# Autodesk Inventor assembly: Z Axis Bed Carrier Assembly
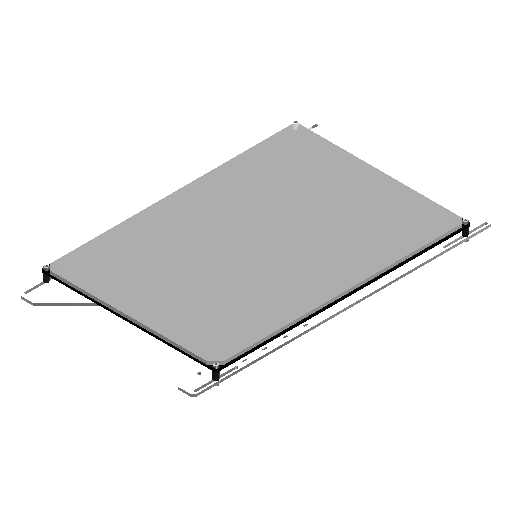
[picture p0: Inventor's stored thumbnail of the model, 512x512]
Saved by Autodesk Inventor 2023.2 (Build 272271000, 271)
## iProperties
Created: 2023-02-18
Part Number: Z Axis Bed Carrier Assembly
Document SubType Name: Assembly
Designer: remop
Author: remop
## Documents named in this file (7)
- C:\Users\remop\OneDrive\Documents\Inventor\3D Printers\LuEVO\Mk5_FullKinematic\Z Axis v2\Z Axis Bed Carrier Assembly.iam
- C:\Users\remop\OneDrive\Documents\Inventor\3D Printers\LuEVO\Mk5_FullKinematic\Z Axis v2\E3D High Temperature Bed 300x200.ipt
- C:\Users\remop\OneDrive\Documents\Inventor\3D Printers\LuEVO\Mk5_FullKinematic\Z Axis v2\Heated Bed Glass.ipt
- C:\Users\remop\OneDrive\Documents\Inventor\3D Printers\LuEVO\Mk5_FullKinematic\Z Axis v2\Bed Carrier.ipt
- C:\Users\remop\OneDrive\Documents\Inventor\3D Printers\LuEVO\Mk5_FullKinematic\Z Axis v2\Heated Bed Spacer.ipt
- C:\Users\remop\OneDrive\Documents\Inventor\3D Printers\LuEVO\Mk5_FullKinematic\XY Motion System\Toolhead\MagToolChanger_CouplerBall.ipt
- C:\Users\remop\OneDrive\Documents\Inventor\Content Center Files\R2023\en-US\AS 1420\AS 1420 - 1973 - M3 x 8.ipt
## Components (18 placed, 6 different names)
1. E3D High Temperature Bed 300x200:1 — Rigid:1, Mate:1, Rigid:2, Rigid:3, Rigid:4, Rigid:5, Insert:1, Insert:2, Insert:6, Insert:8
2. Heated Bed Glass:1 — Rigid:1
3. Bed Carrier:1 — Mate:1, Rigid:6, Rigid:7, Rigid:8
4. Heated Bed Spacer:1 — Rigid:4
5. Heated Bed Spacer:2 — Rigid:2
6. Heated Bed Spacer:3 — Rigid:3
7. Heated Bed Spacer:4 — Rigid:5
8. MagToolChanger_CouplerBall:1 — Rigid:8
9. MagToolChanger_CouplerBall:2 — Rigid:6
10. MagToolChanger_CouplerBall:3 — Rigid:7
11. AS 1420 - Metric M3 x 8:1 — Insert:1
12. AS 1420 - Metric M3 x 8:2 — Insert:2
13. AS 1420 - Metric M3 x 8:6 — Insert:6
14. AS 1420 - Metric M3 x 8:8 — Insert:8
15. AS 1420 - Metric M3 x 8:9
16. AS 1420 - Metric M3 x 8:10
17. AS 1420 - Metric M3 x 8:14
18. AS 1420 - Metric M3 x 8:16
## Relationships (13: WeldJoint 8, Insert 4, Mate 1)
- Rigid:1 [WeldJoint]: E3D High Temperature Bed 300x200:1 ↔ Heated Bed Glass:1
- Mate:1 (10 mm): E3D High Temperature Bed 300x200:1 ↔ Bed Carrier:1
- Rigid:2 [WeldJoint]: E3D High Temperature Bed 300x200:1 ↔ Heated Bed Spacer:2
- Rigid:3 [WeldJoint]: E3D High Temperature Bed 300x200:1 ↔ Heated Bed Spacer:3
- Rigid:4 [WeldJoint]: E3D High Temperature Bed 300x200:1 ↔ Heated Bed Spacer:1
- Rigid:5 [WeldJoint]: E3D High Temperature Bed 300x200:1 ↔ Heated Bed Spacer:4
- Insert:1: E3D High Temperature Bed 300x200:1 ↔ AS 1420 - Metric M3 x 8:1
- Insert:2: E3D High Temperature Bed 300x200:1 ↔ AS 1420 - Metric M3 x 8:2
- Insert:6: E3D High Temperature Bed 300x200:1 ↔ AS 1420 - Metric M3 x 8:6
- Insert:8: E3D High Temperature Bed 300x200:1 ↔ AS 1420 - Metric M3 x 8:8
- Rigid:6 [WeldJoint]: Bed Carrier:1 ↔ MagToolChanger_CouplerBall:2
- Rigid:7 [WeldJoint]: Bed Carrier:1 ↔ MagToolChanger_CouplerBall:3
- Rigid:8 [WeldJoint]: Bed Carrier:1 ↔ MagToolChanger_CouplerBall:1
